# Autodesk Inventor assembly: Drive
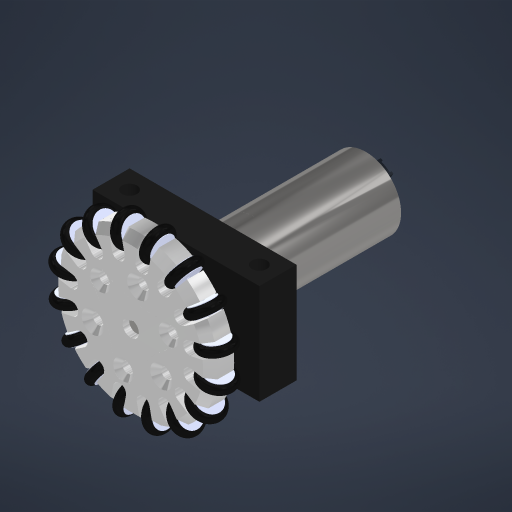
[picture p0: Inventor's stored thumbnail of the model, 512x512]
Saved by Autodesk Inventor 2023 (Build 270158000, 158)
## iProperties
Created: 2023-02-23
Part Number: Drive
Document SubType Name: Assembly
Designer: Elias Braun
Author: Elias Braun
## Documents named in this file (6)
- C:\Users\Elias Braun\Nextcloud2\RoboCup2023\Motor\Drive.iam
- C:\Users\Elias Braun\Nextcloud2\RoboCup2023\Motor\MotorBracket.ipt
- C:\Users\Elias Braun\Nextcloud2\RoboCup2023\Motor\Maxon\B7B9384D898D.iam
- C:\Users\Elias Braun\Nextcloud2\RoboCup2023\Motor\Wheel\Rad.iam
- C:\Users\Elias Braun\Documents\Inventor\Content Center Files\R2023\en-US\BS EN ISO 7046-2 H\BS EN ISO 7046-2 H - M2x5 - 8.8 - H1.ipt
- C:\Users\Elias Braun\Documents\Inventor\Content Center Files\R2023\en-US\DIN 913\DIN 913 - M2,5 x 6.ipt
## Components (7 placed, 5 different names)
1. MotorBracket:1 — Mate:1, Mate:2, Mate:3, Mate:4, Mate:5, Mate:6, Mate:7, Mate:8, Mate:9, Mate:10, Mate:11, Mate:13
2. B7B9384D898D:1 [sub-assembly] — Mate:1, Mate:2, Mate:3, Mate:4, Mate:5, Mate:12
3. Rad:1 [sub-assembly] — Mate:12, Mate:13, Mate:14
4. DIN 913 M2,5 x 6:1 — Mate:14
5. BS EN ISO 7046-2 H M2x5 - 8.8 - H1:3 — Mate:6, Mate:7
6. BS EN ISO 7046-2 H M2x5 - 8.8 - H1:2 — Mate:10, Mate:11
7. BS EN ISO 7046-2 H M2x5 - 8.8 - H1:1 — Mate:8, Mate:9
## Relationships (14: Mate 14)
- Mate:1: MotorBracket:1 ↔ B7B9384D898D:1
- Mate:2: MotorBracket:1 ↔ B7B9384D898D:1
- Mate:3: MotorBracket:1 ↔ B7B9384D898D:1
- Mate:4: MotorBracket:1 ↔ B7B9384D898D:1
- Mate:5: MotorBracket:1 ↔ B7B9384D898D:1
- Mate:6: MotorBracket:1 ↔ BS EN ISO 7046-2 H M2x5 - 8.8 - H1:3
- Mate:7: MotorBracket:1 ↔ BS EN ISO 7046-2 H M2x5 - 8.8 - H1:3
- Mate:8: MotorBracket:1 ↔ BS EN ISO 7046-2 H M2x5 - 8.8 - H1:1
- Mate:9: MotorBracket:1 ↔ BS EN ISO 7046-2 H M2x5 - 8.8 - H1:1
- Mate:10: MotorBracket:1 ↔ BS EN ISO 7046-2 H M2x5 - 8.8 - H1:2
- Mate:11: MotorBracket:1 ↔ BS EN ISO 7046-2 H M2x5 - 8.8 - H1:2
- Mate:12: B7B9384D898D:1 ↔ Rad:1
- Mate:13: MotorBracket:1 ↔ Rad:1
- Mate:14: Rad:1 ↔ DIN 913 M2,5 x 6:1
